# Autodesk Inventor assembly: Assembly_Cube_Lens_holder_v3
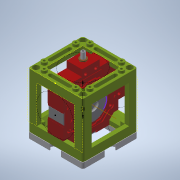
[picture p0: Inventor's stored thumbnail of the model, 180x180]
Saved by Autodesk Inventor 2022 (Build 260153000, 153)
## iProperties
Created: 2020-11-11
Part Number: Assembly_Cube_Lens_holder_v3
Document SubType Name: Assembly
Designer: marsikovabarbora
Author: marsikovabarbora
## Documents named in this file (10)
- G:\My Drive\ASP - M.Sc. Photonics\Practical Modules\MODULE 4 - Master Thesis\2.Experiments\Modules\6.Thorlabs_Pinhole\Assembly_Cube_Pinhole_v3.iam
- G:\My Drive\ASP - M.Sc. Photonics\Practical Modules\MODULE 4 - Master Thesis\2.Experiments\Modules\1.Baseplate\Baseplate_IM\10_Base_puzzle_IM.ipt
- G:\My Drive\ASP - M.Sc. Photonics\Practical Modules\MODULE 4 - Master Thesis\2.Experiments\Modules\2.Base_Cube\Base_Cube_IM\Assembly_Cube_empty_IM_v3.iam
- G:\My Drive\ASP - M.Sc. Photonics\Practical Modules\MODULE 4 - Master Thesis\2.Experiments\Modules\6.Thorlabs_Pinhole\20_Cube_Inser_Flexuremanipulator_m3_screws_v3.ipt
- G:\My Drive\ASP - M.Sc. Photonics\Practical Modules\MODULE 4 - Master Thesis\2.Experiments\Modules\6.Thorlabs_Pinhole\20_Cube_Inser_Flexuremanipulator_springlock_v3.ipt
- G:\My Drive\ASP - M.Sc. Photonics\Practical Modules\MODULE 4 - Master Thesis\2.Experiments\Modules\6.Thorlabs_Pinhole\00_Spring_15mm_6mm.ipt
- G:\My Drive\ASP - M.Sc. Photonics\Practical Modules\MODULE 4 - Master Thesis\2.Experiments\Modules\6.Thorlabs_Pinhole\00_F6SS088-Step.ipt
- G:\My Drive\ASP - M.Sc. Photonics\Practical Modules\MODULE 4 - Master Thesis\2.Experiments\Modules\6.Thorlabs_Pinhole\00_F6SSN2P-Step.ipt
- C:\Users\eda_b\OneDrive\Belgeler\Inventor\Content Center Files\R2022\en-US\DIN 912\DIN 912 - M2 x 0.4 x 10 x 9.ipt
- G:\My Drive\ASP - M.Sc. Photonics\Practical Modules\MODULE 4 - Master Thesis\2.Experiments\Modules\6.Thorlabs_Pinhole\P20K-Step.ipt
## Components (14 placed, 9 different names)
1. Assembly_Cube_empty_IM_v3:1 [sub-assembly] — Rotational:1, Flush:8, Flush:9, Flush:10, Flush:11, Rigid:1
2. 10_Base_puzzle_IM:1 — Rotational:1, Flush:8, Flush:9, Flush:10, Flush:11
3. 20_Cube_Inser_Flexuremanipulator_m3_screws_v3:1 — Rigid:1, Rotational:2, Rigid:2, Rotational:3, Rigid:3, Rotational:4, Rotational:5, Rigid:6, Rigid:7, Rotational:6
4. 20_Cube_Inser_Flexuremanipulator_springlock_v3:1 — Rigid:2
5. 00_Spring_15mm_6mm:1 — Rotational:3
6. 00_F6SS088-Step:1 — Rigid:4
7. 00_F6SSN2P-Step:1 — Rotational:4, Rigid:5
8. 00_Spring_15mm_6mm:2 — Rotational:2
9. 00_F6SS088-Step:2 — Rigid:5
10. 00_F6SSN2P-Step:2 — Rotational:5, Rigid:4
11. 20_Cube_Inser_Flexuremanipulator_springlock_v3:2 — Rigid:3
12. P20K-Step:1 — Rigid:6
13. DIN 912 - replaced by DIN EN ISO 4762 M2 x 10:2 — Rotational:6
14. DIN 912 - replaced by DIN EN ISO 4762 M2 x 10:3 — Rigid:7
## Relationships (22: Flush 8, WeldJoint 7, RevoluteJoint 6, Mate 1)
- [Mate]: Assembly_Cube_empty_IM_v3:1 ↔ 10_Base_puzzle_IM:1
- [Flush]: Assembly_Cube_empty_IM_v3:1 ↔ 10_Base_puzzle_IM:1
- [Flush]: Assembly_Cube_empty_IM_v3:1 ↔ 10_Base_puzzle_IM:1
- [Flush]: Assembly_Cube_empty_IM_v3:1 ↔ 10_Base_puzzle_IM:1
- [Flush]: Assembly_Cube_empty_IM_v3:1 ↔ 10_Base_puzzle_IM:1
- Rotational:1 [RevoluteJoint]: Assembly_Cube_empty_IM_v3:1 ↔ 10_Base_puzzle_IM:1
- Flush:8: Assembly_Cube_empty_IM_v3:1 ↔ 10_Base_puzzle_IM:1
- Flush:9: Assembly_Cube_empty_IM_v3:1 ↔ 10_Base_puzzle_IM:1
- Flush:10: Assembly_Cube_empty_IM_v3:1 ↔ 10_Base_puzzle_IM:1
- Flush:11: Assembly_Cube_empty_IM_v3:1 ↔ 10_Base_puzzle_IM:1
- Rigid:1 [WeldJoint]: Assembly_Cube_empty_IM_v3:1 ↔ 20_Cube_Inser_Flexuremanipulator_m3_screws_v3:1
- Rotational:2 [RevoluteJoint] (-2.5 mm): 20_Cube_Inser_Flexuremanipulator_m3_screws_v3:1 ↔ 00_Spring_15mm_6mm:2
- Rigid:2 [WeldJoint]: 20_Cube_Inser_Flexuremanipulator_m3_screws_v3:1 ↔ 20_Cube_Inser_Flexuremanipulator_springlock_v3:1
- Rotational:3 [RevoluteJoint] (-2 mm): 20_Cube_Inser_Flexuremanipulator_m3_screws_v3:1 ↔ 00_Spring_15mm_6mm:1
- Rigid:3 [WeldJoint]: 20_Cube_Inser_Flexuremanipulator_m3_screws_v3:1 ↔ 20_Cube_Inser_Flexuremanipulator_springlock_v3:2
- Rotational:4 [RevoluteJoint]: 20_Cube_Inser_Flexuremanipulator_m3_screws_v3:1 ↔ 00_F6SSN2P-Step:1
- Rotational:5 [RevoluteJoint]: 20_Cube_Inser_Flexuremanipulator_m3_screws_v3:1 ↔ 00_F6SSN2P-Step:2
- Rigid:4 [WeldJoint] (5 mm): 00_F6SS088-Step:1 ↔ 00_F6SSN2P-Step:2
- Rigid:5 [WeldJoint] (5 mm): 00_F6SSN2P-Step:1 ↔ 00_F6SS088-Step:2
- Rigid:6 [WeldJoint]: 20_Cube_Inser_Flexuremanipulator_m3_screws_v3:1 ↔ P20K-Step:1
- Rigid:7 [WeldJoint] (2.5 mm): 20_Cube_Inser_Flexuremanipulator_m3_screws_v3:1 ↔ DIN 912 - replaced by DIN EN ISO 4762 M2 x 10:3
- Rotational:6 [RevoluteJoint] (-2.5 mm): 20_Cube_Inser_Flexuremanipulator_m3_screws_v3:1 ↔ DIN 912 - replaced by DIN EN ISO 4762 M2 x 10:2
